# Autodesk Inventor assembly: tower_half_mirrored
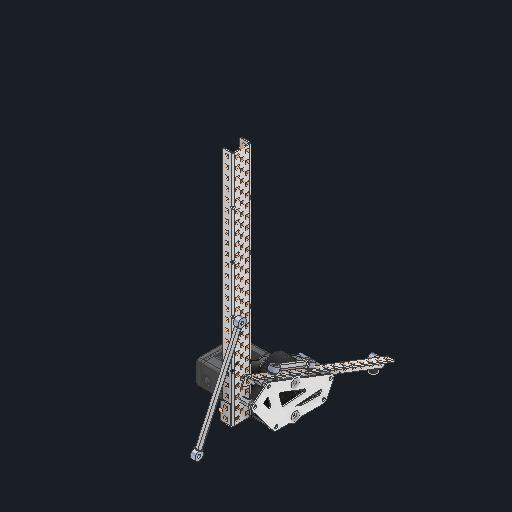
[picture p0: Inventor's stored thumbnail of the model, 512x512]
Saved by Autodesk Inventor 2025 (Build 290162000, 162)
## iProperties
Created: 2024-06-30
Part Number: tower_half_mirrored
Document SubType Name: Assembly
Designer: Averey Ku
Author: Averey Ku
## Documents named in this file (25)
- D:\vex_robotics_high_stakes\hardware\cad\EARLY_SEASON\tower\mirored_parts\tower_half_mirrored.iam
- D:\vex_robotics_high_stakes\hardware\cad\EARLY_SEASON\tower\mirored_parts\Alu C 1x2x1x25_mirrored.ipt
- D:\vex_robotics_high_stakes\hardware\cad\EARLY_SEASON\tower\mirored_parts\Alu C 2x2x2x1_mirrored.ipt
- D:\vex_robotics_high_stakes\hardware\cad\EARLY_SEASON\tower\mirored_parts\C Channel Coupler_mirrored.ipt
- D:\vex_robotics_high_stakes\hardware\cad\EARLY_SEASON\tower\mirored_parts\Shaft Collar No Screw_mirrored.ipt
- D:\vex_robotics_high_stakes\hardware\cad\VEX-CAD-Inventor\Motion\Spacers\Washer Steel\SWasher .375 OD x .015625.ipt
- D:\vex_robotics_high_stakes\hardware\cad\VEX-CAD-Inventor\Motion\Spacers\Washer Steel.ipt
- D:\vex_robotics_high_stakes\hardware\cad\VEX-CAD-Inventor\Structure\Standoff\Standoff 5.00.ipt
- D:\vex_robotics_high_stakes\hardware\cad\VEX-CAD-Inventor\Structure\Standoff.ipt
- D:\vex_robotics_high_stakes\hardware\cad\VEX-CAD-Inventor\Motion\Spacers\Washer Teflon\TWasher .375 OD x .06250.ipt
- D:\vex_robotics_high_stakes\hardware\cad\VEX-CAD-Inventor\Motion\Spacers\Washer Teflon.ipt
- D:\vex_robotics_high_stakes\hardware\cad\EARLY_SEASON\tower\mirored_parts\Alu Angle 1x1x16_mirrored.ipt
- D:\vex_robotics_high_stakes\hardware\cad\VEX-CAD-Inventor\Motion\Spacers\Spacer Nylon .375 OD\NSpacer .375 OD x .125.ipt
- D:\vex_robotics_high_stakes\hardware\cad\VEX-CAD-Inventor\Motion\Spacers\Spacer Nylon .375 OD.ipt
- D:\vex_robotics_high_stakes\hardware\cad\VEX-CAD-Inventor\Motion\Spacers\Spacer Nylon .375 OD\NSpacer .375 OD x .250.ipt
- D:\vex_robotics_high_stakes\hardware\cad\VEX-CAD-Inventor\Motion\Spacers\Washer Teflon\TWasher .375 OD x .04000.ipt
- D:\vex_robotics_high_stakes\hardware\cad\VEX-CAD-Inventor\Motion\Spacers\Washer Teflon\TWasher .375 OD x .03125.ipt
- D:\vex_robotics_high_stakes\hardware\cad\VEX-CAD-Inventor\Motion\Shaft LS\Shaft Collar ipts\Shaft Collar No Screw.ipt
- D:\vex_robotics_high_stakes\hardware\cad\VEX-CAD-Inventor\Structure\Standoff\Standoff 1.50.ipt
- D:\vex_robotics_high_stakes\hardware\cad\VEX-CAD-Inventor\Motion\Shaft HS\HS Pillow Bearing Block.ipt
- D:\vex_robotics_high_stakes\hardware\cad\VEX-CAD-Inventor\Motion\Shaft HS\HS Bushing 0.1250.ipt
- D:\vex_robotics_high_stakes\hardware\cad\EARLY_SEASON\tower\mirored_parts\intake_gearbox_mirrored.iam
- D:\vex_robotics_high_stakes\hardware\cad\VEX-CAD-Inventor\Structure\Hardware\Nut Keps.ipt
- D:\vex_robotics_high_stakes\hardware\cad\VEX-CAD-Inventor\Structure\Hardware\Screw Steel - Star\SScrew Star Smooth 1.500.ipt
- D:\vex_robotics_high_stakes\hardware\cad\VEX-CAD-Inventor\Structure\Hardware\Screw Steel - Star.ipt
## Components (26 placed, 19 different names)
1. Alu C 1x2x1x25_mirrored:1 — Mate:1, Insert:1, Mate:2, Insert:2, Insert:3, Insert:11
2. Alu C 2x2x2x1_mirrored:1 — Mate:1, Insert:1
3. C Channel Coupler_mirrored:1 — Mate:2, Insert:2, Insert:32
4. Shaft Collar No Screw_mirrored:1 — Mate:3, Insert:31
5. SWasher .375 OD x .015625:1 — Insert:5, Insert:31
6. Standoff 5.00:1 — Insert:5, Insert:4
7. Shaft Collar No Screw_mirrored:2 — Insert:4, Mate:3, Insert:3
8. TWasher .375 OD x .06250:1 — Insert:12, Insert:6
9. Alu Angle 1x1x16_mirrored:1 — Insert:12, Insert:11, Mate:4, Insert:16, Insert:17, Insert:20, Mate:7, Mate:8, Insert:33, Insert:34
10. Shaft Collar No Screw_mirrored:3 — Mate:4, Insert:7, Insert:13
11. NSpacer .375 OD x .125:1 — Insert:7, Insert:6
12. NSpacer .375 OD x .250:2 — Insert:10
13. TWasher .375 OD x .04000:2 — Insert:10, Insert:9
14. TWasher .375 OD x .03125:3 — Insert:9, Insert:8
15. SWasher .375 OD x .015625:2 — Insert:13, Insert:8
16. Shaft Collar No Screw:1 — Insert:17, Insert:18
17. Shaft Collar No Screw:2 — Insert:16, Insert:19
18. TWasher .375 OD x .06250:4
19. Standoff 1.50:2
20. NSpacer .375 OD x .125:3 — Insert:19
21. NSpacer .375 OD x .125:4 — Insert:18
22. HS Pillow Bearing Block:1 — Insert:20, Mate:7
23. HS Bushing 0.1250:4
24. intake_gearbox_mirrored:1 [sub-assembly] — Insert:32, Mate:8
25. Nut Keps:1 — Insert:34
26. SScrew Star Smooth 1.500:1 — Insert:33
## Relationships (32: Insert 24, Mate 8)
- Mate:1: Alu C 1x2x1x25_mirrored:1 ↔ Alu C 2x2x2x1_mirrored:1
- Insert:1: Alu C 1x2x1x25_mirrored:1 ↔ Alu C 2x2x2x1_mirrored:1
- Mate:2: Alu C 1x2x1x25_mirrored:1 ↔ C Channel Coupler_mirrored:1
- Insert:2: Alu C 1x2x1x25_mirrored:1 ↔ C Channel Coupler_mirrored:1
- Insert:5: SWasher .375 OD x .015625:1 ↔ Standoff 5.00:1
- Insert:4: Standoff 5.00:1 ↔ Shaft Collar No Screw_mirrored:2
- Mate:3: Shaft Collar No Screw_mirrored:1 ↔ Shaft Collar No Screw_mirrored:2
- Insert:3: Alu C 1x2x1x25_mirrored:1 ↔ Shaft Collar No Screw_mirrored:2
- Insert:12: TWasher .375 OD x .06250:1 ↔ Alu Angle 1x1x16_mirrored:1
- Insert:11: Alu C 1x2x1x25_mirrored:1 ↔ Alu Angle 1x1x16_mirrored:1
- Mate:4: Alu Angle 1x1x16_mirrored:1 ↔ Shaft Collar No Screw_mirrored:3
- Insert:7: Shaft Collar No Screw_mirrored:3 ↔ NSpacer .375 OD x .125:1
- Insert:6: TWasher .375 OD x .06250:1 ↔ NSpacer .375 OD x .125:1
- Insert:10: NSpacer .375 OD x .250:2 ↔ TWasher .375 OD x .04000:2
- Insert:9: TWasher .375 OD x .04000:2 ↔ TWasher .375 OD x .03125:3
- Insert:13: Shaft Collar No Screw_mirrored:3 ↔ SWasher .375 OD x .015625:2
- Insert:8: TWasher .375 OD x .03125:3 ↔ SWasher .375 OD x .015625:2
- [Mate]: Shaft Collar No Screw:1 ↔ Shaft Collar No Screw:2
- [Mate]: Shaft Collar No Screw:1 ↔ Shaft Collar No Screw:2
- [Insert]: Shaft Collar No Screw:1 ↔ TWasher .375 OD x .06250:4
- [Insert]: TWasher .375 OD x .06250:4 ↔ Standoff 1.50:2
- Insert:16 (3.175 mm): Alu Angle 1x1x16_mirrored:1 ↔ Shaft Collar No Screw:2
- Insert:17 (3.175 mm): Alu Angle 1x1x16_mirrored:1 ↔ Shaft Collar No Screw:1
- Insert:18: Shaft Collar No Screw:1 ↔ NSpacer .375 OD x .125:4
- Insert:19: Shaft Collar No Screw:2 ↔ NSpacer .375 OD x .125:3
- Insert:20: Alu Angle 1x1x16_mirrored:1 ↔ HS Pillow Bearing Block:1
- Mate:7: Alu Angle 1x1x16_mirrored:1 ↔ HS Pillow Bearing Block:1
- Insert:31 (0.1385 mm): Shaft Collar No Screw_mirrored:1 ↔ SWasher .375 OD x .015625:1
- Insert:32 (12.7 mm): C Channel Coupler_mirrored:1 ↔ intake_gearbox_mirrored:1
- Mate:8: Alu Angle 1x1x16_mirrored:1 ↔ intake_gearbox_mirrored:1
- Insert:33: Alu Angle 1x1x16_mirrored:1 ↔ SScrew Star Smooth 1.500:1
- Insert:34: Alu Angle 1x1x16_mirrored:1 ↔ Nut Keps:1
